# Autodesk Inventor assembly: Chuck Assembly
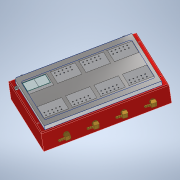
[picture p0: Inventor's stored thumbnail of the model, 180x180]
Saved by Autodesk Inventor 2022 (Build 260153000, 153)
## iProperties
Created: 2021-01-11
Part Number: Chuck Assembly
Document SubType Name: Assembly
Designer: caleb
Author: caleb
## Documents named in this file (5)
- C:\Users\Caleb\Desktop\nebraska-silicon-lab\Hardware\ETL\Module Assembly\Chuck - Octopocket\Chuck - Octopocket.iam
- C:\Users\Caleb\Desktop\nebraska-silicon-lab\Hardware\ETL\Module Assembly\Chuck - Octopocket\90128A212_ZNC-PLTD ALLOY STL SCKT HEAD CAP SCREW.ipt
- C:\Users\Caleb\Desktop\nebraska-silicon-lab\Hardware\ETL\Module Assembly\Chuck - Octopocket\44555K147_BRASS BARBED TUBE FITTING FOR VACUUM.ipt
- C:\Users\Caleb\Desktop\nebraska-silicon-lab\Hardware\ETL\Module Assembly\Chuck - Octopocket\Chuck - Octopocket.ipt
- C:\Users\Caleb\Desktop\nebraska-silicon-lab\Hardware\ETL\Module Assembly\BBM Staging Plate\BBM Staging Plate Assembly.iam
## Components (13 placed, 4 different names)
1. Chuck - Octopocket:1 — Insert:1, Insert:2, Insert:3, Insert:6, Insert:7, Insert:8, Insert:9, Insert:10, Insert:11, Insert:12, Insert:13, Mate:1, Angle:1
2. 90128A212_ZNC-PLTD ALLOY STL SCKT HEAD CAP SCREW:1 — Insert:2, Tangent:2
3. 90128A212_ZNC-PLTD ALLOY STL SCKT HEAD CAP SCREW:2 — Insert:3
4. 90128A212_ZNC-PLTD ALLOY STL SCKT HEAD CAP SCREW:3 — Insert:1, Tangent:1
5. 44555K147_BRASS BARBED TUBE FITTING FOR VACUUM:1 — Insert:7
6. 44555K147_BRASS BARBED TUBE FITTING FOR VACUUM:2 — Insert:10
7. 44555K147_BRASS BARBED TUBE FITTING FOR VACUUM:3 — Insert:11
8. 44555K147_BRASS BARBED TUBE FITTING FOR VACUUM:4 — Insert:12
9. 44555K147_BRASS BARBED TUBE FITTING FOR VACUUM:5 — Insert:13
10. 44555K147_BRASS BARBED TUBE FITTING FOR VACUUM:6 — Insert:9
11. 44555K147_BRASS BARBED TUBE FITTING FOR VACUUM:7 — Insert:8
12. 44555K147_BRASS BARBED TUBE FITTING FOR VACUUM:8 — Insert:6
13. BBM Staging Plate Assembly:1 [sub-assembly] — Mate:1, Angle:1, Tangent:1, Tangent:2
## Relationships (15: Insert 11, Tangent 2, Mate 1, Angle 1)
- Insert:1: Chuck - Octopocket:1 ↔ 90128A212_ZNC-PLTD ALLOY STL SCKT HEAD CAP SCREW:3
- Insert:2: Chuck - Octopocket:1 ↔ 90128A212_ZNC-PLTD ALLOY STL SCKT HEAD CAP SCREW:1
- Insert:3: Chuck - Octopocket:1 ↔ 90128A212_ZNC-PLTD ALLOY STL SCKT HEAD CAP SCREW:2
- Insert:6: Chuck - Octopocket:1 ↔ 44555K147_BRASS BARBED TUBE FITTING FOR VACUUM:8
- Insert:7: Chuck - Octopocket:1 ↔ 44555K147_BRASS BARBED TUBE FITTING FOR VACUUM:1
- Insert:8: Chuck - Octopocket:1 ↔ 44555K147_BRASS BARBED TUBE FITTING FOR VACUUM:7
- Insert:9: Chuck - Octopocket:1 ↔ 44555K147_BRASS BARBED TUBE FITTING FOR VACUUM:6
- Insert:10: Chuck - Octopocket:1 ↔ 44555K147_BRASS BARBED TUBE FITTING FOR VACUUM:2
- Insert:11: Chuck - Octopocket:1 ↔ 44555K147_BRASS BARBED TUBE FITTING FOR VACUUM:3
- Insert:12: Chuck - Octopocket:1 ↔ 44555K147_BRASS BARBED TUBE FITTING FOR VACUUM:4
- Insert:13: Chuck - Octopocket:1 ↔ 44555K147_BRASS BARBED TUBE FITTING FOR VACUUM:5
- Mate:1: Chuck - Octopocket:1 ↔ BBM Staging Plate Assembly:1
- Angle:1 (0 deg): Chuck - Octopocket:1 ↔ BBM Staging Plate Assembly:1
- Tangent:1: 90128A212_ZNC-PLTD ALLOY STL SCKT HEAD CAP SCREW:3 ↔ BBM Staging Plate Assembly:1
- Tangent:2: 90128A212_ZNC-PLTD ALLOY STL SCKT HEAD CAP SCREW:1 ↔ BBM Staging Plate Assembly:1
